# Autodesk Inventor assembly: hubRings
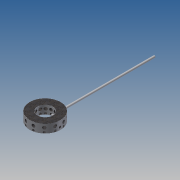
[picture p0: Inventor's stored thumbnail of the model, 180x180]
Saved by Autodesk Inventor 2014 SP1 (Build 180222100, 222)
## iProperties
Created: 2014-12-02
Part Number: hubRings
Document SubType Name: Assembly
Designer: Dave
Author: Dave
## Documents named in this file (5)
- C:\Users\Dave\Desktop\hera-cad\hub\hubRings.iam
- C:\Users\Dave\Desktop\hera-cad\hub\ringInner.ipt
- C:\Users\Dave\Desktop\hera-cad\hub\ringOuter.ipt
- C:\Users\Dave\Desktop\hera-cad\hub\cement.ipt
- C:\Users\Dave\Desktop\hera-cad\support\sparHoriz.ipt
## Components (4 placed, 4 different names)
1. ringInner:1 — Angle:1, Insert:1, Insert:2
2. ringOuter:1 — Angle:1, Insert:1
3. cement:1 — Insert:2
4. sparHoriz:1
## Relationships (3: Insert 2, Angle 1)
- Angle:1 (0 deg): ringInner:1 ↔ ringOuter:1
- Insert:1: ringInner:1 ↔ ringOuter:1
- Insert:2: ringInner:1 ↔ cement:1
